# Autodesk Inventor assembly: SirHexAlot
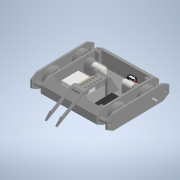
[picture p0: Inventor's stored thumbnail of the model, 180x180]
Saved by Autodesk Inventor 2020 (Build 240168000, 168)
## iProperties
Created: 2023-12-21
Part Number: SirHexAlot
Document SubType Name: Assembly
Designer: smz3rm
Mass: 450.2 g
Surface Area: 1649.78 cm^2
Volume: 365.309 cm^3
Density: 1.23238 g/cm^3
Author: smz3rm
## Documents named in this file (14)
- C:\Users\smz3rm\OneDrive - BP\Documents\DigitalTwin\Models\BattleBot\Flipper\SirHexAlot.iam
- C:\Users\smz3rm\OneDrive - BP\Documents\DigitalTwin\Models\BattleBot\Flipper\HexBody.ipt
- C:\Users\smz3rm\OneDrive - BP\Documents\DigitalTwin\Models\BattleBot\Flipper\HexWheelGuard.ipt
- C:\Users\smz3rm\OneDrive - BP\Documents\DigitalTwin\Models\BattleBot\Flipper\PulleyedWheelV1.ipt
- C:\Users\smz3rm\OneDrive - BP\Documents\DigitalTwin\Models\BattleBot\DriveMotorV2.ipt
- C:\Users\smz3rm\OneDrive - BP\Documents\DigitalTwin\Models\BattleBot\SwitchHolder.ipt
- C:\Users\smz3rm\OneDrive - BP\Documents\DigitalTwin\Models\BattleBot\Switch.ipt
- C:\Users\smz3rm\OneDrive - BP\Documents\DigitalTwin\Models\BattleBot\BatteryV1.ipt
- C:\Users\smz3rm\OneDrive - BP\Documents\DigitalTwin\Models\BattleBot\Flipper\Servo.ipt
- C:\Users\smz3rm\OneDrive - BP\Documents\DigitalTwin\Models\BattleBot\Flipper\PulleyedBearingWheelV1.ipt
- C:\Users\smz3rm\OneDrive - BP\Documents\DigitalTwin\Models\BattleBot\Flipper\WheelBearings.ipt
- C:\Users\smz3rm\OneDrive - BP\Documents\DigitalTwin\Models\BattleBot\Flipper\FlipperRod.ipt
- C:\Users\smz3rm\OneDrive - BP\Documents\DigitalTwin\Models\BattleBot\Flipper\HexFlipper.ipt
- C:\Users\smz3rm\OneDrive - BP\Documents\DigitalTwin\Models\BattleBot\Flipper\HexFlipperSpike.ipt
## Components (21 placed, 13 different names)
1. HexBody:1 — Mate:3, Mate:4, Mate:5, Mate:6, Mate:7, Mate:8, Mate:9, Mate:11, Mate:14, Mate:22, Mate:23, Mate:24, Mate:29, Mate:30, Mate:39, Mate:41, Mate:42, Mate:44, Mate:45, Mate:46, Mate:47, Mate:48, Mate:51, Mate:52, Mate:53
2. HexWheelGuard:1 — Mate:25, Mate:29, Mate:43, Mate:44, Mate:45
3. PulleyedWheelV1:1 — Mate:10, Mate:11
4. DriveMotorV2:1 — Mate:7, Mate:8, Mate:9, Mate:10, Mate:25
5. DriveMotorV2:2 — Mate:4, Mate:5, Mate:6, Mate:15, Mate:27
6. SwitchHolder:1 — Mate:19, Mate:20, Mate:21, Mate:22, Mate:23
7. Switch:1 — Mate:19, Mate:20, Mate:21
8. BatteryV1:1 — Mate:24, Mate:52, Mate:53
9. PulleyedWheelV1:5 — Mate:14, Mate:15
10. HexWheelGuard:2 — Mate:27, Mate:30, Mate:40, Mate:46, Mate:47
11. Servo:1 — Mate:3
12. PulleyedBearingWheelV1:1 — Mate:31, Mate:32, Mate:33, Mate:34, Mate:42
13. PulleyedBearingWheelV1:2 — Mate:35, Mate:36, Mate:37, Mate:38, Mate:39
14. WheelBearings:1 — Mate:31, Mate:32, Mate:43
15. WheelBearings:2 — Mate:33, Mate:34, Mate:41
16. WheelBearings:3 — Mate:35, Mate:36
17. WheelBearings:4 — Mate:37, Mate:38, Mate:40
18. FlipperRod:1 — Mate:49, Mate:50
19. HexFlipper:1 — Mate:49, Mate:50, Mate:51, Mate:54, Mate:55, Mate:56, Mate:57, Mate:58, Mate:59
20. HexFlipperSpike:1 — Mate:57, Mate:58, Mate:59
21. HexFlipperSpike:2 — Mate:54, Mate:55, Mate:56
## Relationships (50: Mate 50)
- Mate:3: HexBody:1 ↔ Servo:1
- Mate:4: HexBody:1 ↔ DriveMotorV2:2
- Mate:5: HexBody:1 ↔ DriveMotorV2:2
- Mate:6: HexBody:1 ↔ DriveMotorV2:2
- Mate:7: HexBody:1 ↔ DriveMotorV2:1
- Mate:8: HexBody:1 ↔ DriveMotorV2:1
- Mate:9: HexBody:1 ↔ DriveMotorV2:1
- Mate:10: PulleyedWheelV1:1 ↔ DriveMotorV2:1
- Mate:11: HexBody:1 ↔ PulleyedWheelV1:1
- Mate:14: HexBody:1 ↔ PulleyedWheelV1:5
- Mate:15: DriveMotorV2:2 ↔ PulleyedWheelV1:5
- Mate:19: SwitchHolder:1 ↔ Switch:1
- Mate:20: SwitchHolder:1 ↔ Switch:1
- Mate:21: SwitchHolder:1 ↔ Switch:1
- Mate:22: HexBody:1 ↔ SwitchHolder:1
- Mate:23: HexBody:1 ↔ SwitchHolder:1
- Mate:24: HexBody:1 ↔ BatteryV1:1
- Mate:25: HexWheelGuard:1 ↔ DriveMotorV2:1
- Mate:27: DriveMotorV2:2 ↔ HexWheelGuard:2
- Mate:29: HexBody:1 ↔ HexWheelGuard:1
- Mate:30: HexBody:1 ↔ HexWheelGuard:2
- Mate:31: PulleyedBearingWheelV1:1 ↔ WheelBearings:1
- Mate:32: PulleyedBearingWheelV1:1 ↔ WheelBearings:1
- Mate:33: PulleyedBearingWheelV1:1 ↔ WheelBearings:2
- Mate:34: PulleyedBearingWheelV1:1 ↔ WheelBearings:2
- Mate:35: PulleyedBearingWheelV1:2 ↔ WheelBearings:3
- Mate:36: PulleyedBearingWheelV1:2 ↔ WheelBearings:3
- Mate:37: PulleyedBearingWheelV1:2 ↔ WheelBearings:4
- Mate:38: PulleyedBearingWheelV1:2 ↔ WheelBearings:4
- Mate:39: HexBody:1 ↔ PulleyedBearingWheelV1:2
- Mate:40: HexWheelGuard:2 ↔ WheelBearings:4
- Mate:41: HexBody:1 ↔ WheelBearings:2
- Mate:42: HexBody:1 ↔ PulleyedBearingWheelV1:1
- Mate:43: HexWheelGuard:1 ↔ WheelBearings:1
- Mate:44: HexBody:1 ↔ HexWheelGuard:1
- Mate:45: HexBody:1 ↔ HexWheelGuard:1
- Mate:46: HexBody:1 ↔ HexWheelGuard:2
- Mate:47: HexBody:1 ↔ HexWheelGuard:2
- Mate:48: HexBody:1
- Mate:49: FlipperRod:1 ↔ HexFlipper:1
- Mate:50: FlipperRod:1 ↔ HexFlipper:1
- Mate:51: HexBody:1 ↔ HexFlipper:1
- Mate:52: HexBody:1 ↔ BatteryV1:1
- Mate:53: HexBody:1 ↔ BatteryV1:1
- Mate:54: HexFlipper:1 ↔ HexFlipperSpike:2
- Mate:55: HexFlipper:1 ↔ HexFlipperSpike:2
- Mate:56: HexFlipper:1 ↔ HexFlipperSpike:2
- Mate:57: HexFlipper:1 ↔ HexFlipperSpike:1
- Mate:58: HexFlipper:1 ↔ HexFlipperSpike:1
- Mate:59: HexFlipper:1 ↔ HexFlipperSpike:1
